# Autodesk Inventor assembly: FluteMelodicaAssembly0
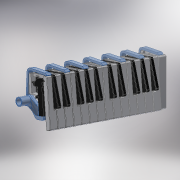
[picture p0: Inventor's stored thumbnail of the model, 180x180]
Saved by Autodesk Inventor 2018 (Build 220112000, 112)
## iProperties
Created: 2018-10-12
Part Number: FluteMelodicaAssembly0
Document SubType Name: Assembly
Designer: Isaac Newcomb
Mass: 621.941 g
Surface Area: 3691.55 cm^2
Volume: 586.736 cm^3
Density: 1.06 g/cm^3
Author: Isaac Newcomb
## Documents named in this file (15)
- E:\ICE KEYS\IceKeysAssembly0.iam
- E:\ICE KEYS\PostValve1.ipt
- E:\ICE KEYS\Manifold2.ipt
- E:\ICE KEYS\CKey0.ipt
- E:\ICE KEYS\BlackKey1.ipt
- E:\ICE KEYS\DKey0.ipt
- E:\ICE KEYS\EKey0.ipt
- E:\ICE KEYS\FKey0.ipt
- E:\ICE KEYS\GKey0.ipt
- E:\ICE KEYS\AKey0.ipt
- E:\ICE KEYS\BKey0.ipt
- E:\ICE KEYS\TopCKey0.ipt
- E:\ICE KEYS\ManifoldExtension2.ipt
- E:\ICE KEYS\HousingArm0.ipt
- E:\ICE KEYS\PostValveLast0.ipt
## Components (39 placed, 14 different names)
1. Manifold2:1 — Rigid:1, Rigid:2, Rigid:3
2. ManifoldExtension2:1 — Rigid:2
3. TopCKey0:1
4. PostValveLast0:1 — Rigid:4
5. PostValve1:1 — Rigid:1, Rotational:1, Rotational:2, Rotational:3, Rotational:4
6. PostValve1:3 — Rotational:5, Rotational:6, Rotational:7, Rotational:8
7. PostValve1:4 — Rotational:9
8. PostValve1:5 — Rigid:4
9. CKey0:1 — Rotational:1
10. CKey0:2
11. DKey0:1 — Rotational:3
12. DKey0:2
13. EKey0:1 — Rotational:4
14. EKey0:2
15. FKey0:1 — Rotational:5
16. FKey0:2
17. GKey0:1 — Rotational:7
18. GKey0:2
19. AKey0:1 — Rotational:8
20. AKey0:2
21. BKey0:1 — Rotational:9
22. BKey0:2
23. HousingArm0:1 — Rigid:3
24. HousingArm0:2
25. HousingArm0:3
26. HousingArm0:4
27. HousingArm0:5
28. HousingArm0:6
29. HousingArm0:7
30. BlackKey1:1 — Rotational:2
31. BlackKey1:2
32. BlackKey1:3
33. BlackKey1:4
34. BlackKey1:5 — Rotational:6
35. BlackKey1:6
36. BlackKey1:7
37. BlackKey1:8
38. BlackKey1:9
39. BlackKey1:10
## Component patterns: (4 elements, first: PostValve1:1), (2 elements, first: CKey0:1), (2 elements, first: DKey0:1), (2 elements), (2 elements, first: EKey0:1), (2 elements, first: FKey0:1), (3 elements), (2 elements, first: GKey0:1), (2 elements, first: AKey0:1), (2 elements, first: BKey0:1), (7 elements, first: HousingArm0:1), (2 elements, first: BlackKey1:1), Component Pattern 17:2 (2 elements), (2 elements, first: BlackKey1:5), Component Pattern 23:2 (2 elements), Component Pattern 23:3 (2 elements)
## Relationships (13: RevoluteJoint 9, WeldJoint 4)
- Rigid:1 [WeldJoint]: Manifold2:1 ↔ PostValve1:1
- Rotational:1 [RevoluteJoint]: PostValve1:1 ↔ CKey0:1
- Rotational:2 [RevoluteJoint]: PostValve1:1 ↔ BlackKey1:1
- Rotational:3 [RevoluteJoint]: PostValve1:1 ↔ DKey0:1
- Rotational:4 [RevoluteJoint]: PostValve1:1 ↔ EKey0:1
- Rotational:5 [RevoluteJoint]: PostValve1:3 ↔ FKey0:1
- Rotational:6 [RevoluteJoint]: PostValve1:3 ↔ BlackKey1:5
- Rotational:7 [RevoluteJoint]: PostValve1:3 ↔ GKey0:1
- Rotational:8 [RevoluteJoint]: PostValve1:3 ↔ AKey0:1
- Rotational:9 [RevoluteJoint]: PostValve1:4 ↔ BKey0:1
- Rigid:2 [WeldJoint]: Manifold2:1 ↔ ManifoldExtension2:1
- Rigid:3 [WeldJoint]: Manifold2:1 ↔ HousingArm0:1
- Rigid:4 [WeldJoint]: PostValveLast0:1 ↔ PostValve1:5
## Named parameters: KeyCount = 25, KeyWidth = 10 mm, KeySpacing = 0.5 mm
